# Autodesk Inventor assembly: emsamble caja
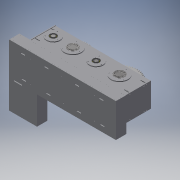
[picture p0: Inventor's stored thumbnail of the model, 180x180]
Saved by Autodesk Inventor 2018 (Build 220112000, 112)
## iProperties
Created: 2017-08-31
Part Number: emsamble caja
Material: Genérico
Document SubType Name: Assembly
Designer: Alumno
Author: Alumno
## Documents named in this file (34)
- C:\Users\isai\Documents\GitHub\caja-reductora-II\emsamble caja.iam
- C:\Users\isai\Documents\GitHub\caja-reductora-II\EJE 2 (30 mm y 15 mm).iam
- C:\Users\isai\Documents\GitHub\caja-reductora-II\TREN 1\Design Accelerator\Engranaje recto12.ipt
- C:\Users\isai\Documents\GitHub\caja-reductora-II\TREN 1\Design Accelerator\Engranaje recto22.ipt
- C:\Users\isai\Documents\GitHub\caja-reductora-II\TREN 2\Design Accelerator\Engranaje recto11.ipt
- C:\Users\isai\Documents\GitHub\caja-reductora-II\TREN 2\Design Accelerator\Engranaje recto21.ipt
- C:\Users\isai\Documents\GitHub\caja-reductora-II\TREN 3\Design Accelerator\Engranaje recto11.ipt
- C:\Users\isai\Documents\GitHub\caja-reductora-II\TREN 3\Design Accelerator\Engranaje recto21.ipt
- C:\Users\isai\Documents\GitHub\caja-reductora-II\EJE 3 (30-45).iam
- C:\Users\isai\Documents\GitHub\caja-reductora-II\EJE 4.iam
- C:\Users\isai\Documents\GitHub\caja-reductora-II\Chaveta- Tren 1.ipt
- C:\Users\isai\Documents\GitHub\caja-reductora-II\Chaveta 25.ipt
- C:\Users\isai\Documents\GitHub\caja-reductora-II\EJE 1.iam
- C:\Users\isai\Documents\GitHub\caja-reductora-II\RODAMIENTO 15 D\6002.iam
- C:\Users\isai\Documents\GitHub\caja-reductora-II\RODAMIENTO 25 D\6005.iam
- C:\Users\isai\Documents\GitHub\caja-reductora-II\ACO.RODA15.ipt
- C:\Users\isai\Documents\GitHub\caja-reductora-II\ACO.RODA25.ipt
- C:\Users\isai\Documents\GitHub\caja-reductora-II\P1.ipt
- C:\Users\isai\Documents\GitHub\caja-reductora-II\P2.ipt
- C:\Users\isai\Documents\GitHub\caja-reductora-II\P3.ipt
- C:\Users\isai\Documents\GitHub\caja-reductora-II\MOTOR DC.ipt
- C:\Users\isai\Documents\Inventor\Content Center Files\R2018\en-US\GB_T 29.1\Bolt GB_T 29.1 M3 x 25.ipt
- C:\Users\isai\Documents\GitHub\caja-reductora-II\SUPORT STEEP.ipt
- C:\Users\isai\Documents\GitHub\caja-reductora-II\SUPORT STEEP 2.ipt
- C:\Users\isai\Documents\Inventor\Content Center Files\R2018\en-US\AS 1112 (2)\AS 1112 - M3  Type 5.ipt
- C:\Users\isai\Documents\Inventor\Content Center Files\R2018\en-US\GB_T 29.1\Bolt GB_T 29.1 M3 x 16.ipt
- C:\Users\isai\Documents\GitHub\caja-reductora-II\PISO.ipt
- C:\Users\isai\Documents\GitHub\caja-reductora-II\FLOOR.ipt
- C:\Users\isai\Documents\GitHub\caja-reductora-II\F1.ipt
- C:\Users\isai\Documents\GitHub\caja-reductora-II\F2.ipt
- C:\Users\isai\Documents\GitHub\caja-reductora-II\F3.ipt
- C:\Users\isai\Documents\GitHub\caja-reductora-II\F4.ipt
- C:\Users\isai\Documents\GitHub\caja-reductora-II\F6.ipt
- C:\Users\isai\Documents\GitHub\caja-reductora-II\F7.ipt
## Components (60 placed, 29 different names)
1. Engranaje recto1:1 — Coincidencia:1, Ángulo:2, Coincidencia:16
2. Engranaje recto2:1 — Coincidencia:5, Coincidencia:6, Ángulo:2, Coincidencia:17
3. Engranaje recto2:2 — Mate:32, Mate:33
4. Engranaje recto1:3 — Mate:27, Mate:30, Mate:40, Mate:51
5. Engranaje recto2:3 — Mate:28, Mate:29
6. EJE 2 (30 mm y 15 mm):3 [sub-assembly] — Coincidencia:2, Coincidencia:3, Coincidencia:4, Coincidencia:5, Ángulo:1, Ángulo:3, Coincidencia:17, Nivelación:1, Mate:31, Mate:34, Mate:36, Mate:41, Mate:44, Mate:56, Mate:59
7. Engranaje recto1:4 — Mate:31, Mate:34, Mate:38, Mate:53
8. EJE 3 (30-45):1 [sub-assembly] — Coincidencia:9, Coincidencia:10, Coincidencia:11, Ángulo:3, Ángulo:4, Nivelación:2, Nivelación:3, Mate:27, Mate:30, Mate:32, Mate:33, Mate:39, Mate:47, Mate:48, Mate:54, Mate:60
9. EJE 4:1 [sub-assembly] — Coincidencia:19, Coincidencia:20, Coincidencia:21, Ángulo:4, Nivelación:3, Mate:28, Mate:29, Mate:42, Mate:43, Mate:49, Mate:55, Mate:57, Mate:61, Mate:64
10. Chaveta- Tren 1:1 — Coincidencia:2, Coincidencia:3, Coincidencia:4, Coincidencia:6
11. Chaveta- Tren 1:2 — Coincidencia:19, Coincidencia:20, Coincidencia:21
12. Chaveta 25:6 — Coincidencia:9, Coincidencia:10, Coincidencia:11
13. EJE 1:1 [sub-assembly] — Coincidencia:1, Ángulo:1, Coincidencia:16, Nivelación:1, Nivelación:2, Mate:35, Mate:45, Mate:46, Mate:50, Mate:52, Mate:58, Mate:63, Mate:89
14. 6002:6 [sub-assembly] — Mate:35, Mate:45, Flush:6
15. 6002:7 [sub-assembly] — Mate:46, Flush:5, Flush:8
16. 6002:8 [sub-assembly] — Mate:36, Mate:38, Flush:9
17. 6002:9 [sub-assembly] — Mate:39, Mate:40, Flush:7
18. 6005:1 [sub-assembly] — Mate:42, Mate:43, Flush:11
19. 6005:2 [sub-assembly] — Mate:47, Mate:48, Flush:4, Flush:5, Flush:12
20. 6005:3 [sub-assembly] — Mate:41, Mate:44, Flush:13
21. 6005:4 [sub-assembly] — Mate:49, Flush:4, Flush:10
22. ACO.RODA15:1 — Mate:50, Flush:6, Mate:62
23. ACO.RODA15:2 — Mate:51, Flush:7
24. ACO.RODA15:3 — Mate:52, Flush:8, Mate:70, Mate:72, Mate:97
25. ACO.RODA15:4 — Mate:53, Flush:9
26. ACO.RODA25:1 — Mate:54, Flush:12
27. ACO.RODA25:2 — Mate:57, Flush:10, Mate:65
28. ACO.RODA25:3 — Mate:56, Flush:13
29. ACO.RODA25:4 — Mate:55, Flush:11
30. P1:1 — Mate:58, Mate:59, Mate:60, Mate:61, Mate:62, Flush:14, Mate:67, Flush:15, Mate:112, Mate:113, Mate:114, Mate:115, Mate:116, Flush:23
31. P2:1 — Mate:63, Mate:64, Mate:65, Mate:66, Mate:71, Mate:73, Mate:74
32. P3:1 — Mate:66, Flush:14, Angle:5
33. P3:2 — Mate:67, Flush:15, Angle:6
34. MOTOR DC:1 — Mate:89, Angle:5, Mate:90, Mate:91
35. Bolt GB/T 29.1 M3x25:2 — Mate:70, Mate:71, Mate:74, Mate:84, Mate:85, Flush:16, Flush:18
36. Bolt GB/T 29.1 M3x25:3 — Mate:72, Mate:73, Mate:75, Mate:86, Flush:17
37. SUPORT STEEP:1 — Mate:75, Mate:84, Mate:88, Mate:99, Mate:100, Mate:101, Mate:102, Mate:104
38. AS 1112 (2) - Metric M3  Type 5:1 — Mate:85, Flush:16, Mate:88
39. AS 1112 (2) - Metric M3  Type 5:2 — Mate:86, Flush:17
40. AS 1112 (2) - Metric M3  Type 5:3 — Mate:98, Flush:19
41. SUPORT STEEP 2:1 — Mate:90, Mate:91, Mate:103, Mate:108, Mate:109, Mate:110, Mate:111
42. Bolt GB/T 29.1 M3x25:4 — Mate:97, Flush:18, Mate:98, Flush:19
43. Bolt GB/T 29.1 M3x25:5 — Mate:99, Mate:101, Mate:107, Flush:22
44. Bolt GB/T 29.1 M3x25:6 — Mate:100, Mate:102, Mate:106, Flush:21
45. Bolt GB/T 29.1 M3x25:7 — Mate:103, Mate:104, Mate:105, Flush:20
46. AS 1112 (2) - Metric M3  Type 5:4 — Mate:105, Flush:20
47. AS 1112 (2) - Metric M3  Type 5:5
48. AS 1112 (2) - Metric M3  Type 5:6 — Mate:106, Flush:21
49. AS 1112 (2) - Metric M3  Type 5:7 — Mate:107, Flush:22
50. Bolt GB/T 29.1 M3x16:1 — Mate:108, Mate:109
51. Bolt GB/T 29.1 M3x16:2 — Mate:110, Mate:111
52. PISO:1 — Mate:112, Mate:113, Mate:114
53. FLOOR:1 — Angle:6, Mate:115, Mate:116, Flush:23, Mate:117, Flush:24, Mate:118, Mate:119, Flush:25, Flush:26, Mate:120, Flush:27, Flush:28, Mate:121, Flush:29, Flush:30, Mate:122, Flush:31, Flush:32, Mate:123, Flush:33, Flush:34
54. F1:1 — Mate:117, Flush:24, Mate:118
55. F2:1 — Mate:119, Flush:25, Flush:26
56. F3:1 — Mate:120, Flush:27, Flush:28
57. F4:1 — Mate:121, Flush:29, Flush:30, Mate:124, Mate:125, Flush:35
58. F6:1 — Mate:122, Flush:31, Flush:32
59. F7:1 — Mate:123, Flush:33, Flush:34
60. FLOOR:2 — Mate:124, Mate:125, Flush:35
## Relationships (137: Mate 96, Flush 35, Angle 6)
- Coincidencia:1 [Mate]: Engranaje recto1:1 ↔ EJE 1:1
- Coincidencia:2 [Mate]: EJE 2 (30 mm y 15 mm):3 ↔ Chaveta- Tren 1:1
- Coincidencia:3 [Mate]: EJE 2 (30 mm y 15 mm):3 ↔ Chaveta- Tren 1:1
- Coincidencia:4 [Mate]: EJE 2 (30 mm y 15 mm):3 ↔ Chaveta- Tren 1:1
- Coincidencia:5 [Mate]: Engranaje recto2:1 ↔ EJE 2 (30 mm y 15 mm):3
- Coincidencia:6 [Mate]: Engranaje recto2:1 ↔ Chaveta- Tren 1:1
- Ángulo:1 [Angle] (0 deg): EJE 2 (30 mm y 15 mm):3 ↔ EJE 1:1
- Ángulo:2 [Angle] (0 deg): Engranaje recto1:1 ↔ Engranaje recto2:1
- Coincidencia:9 [Mate]: EJE 3 (30-45):1 ↔ Chaveta 25:6
- Coincidencia:10 [Mate]: EJE 3 (30-45):1 ↔ Chaveta 25:6
- Coincidencia:11 [Mate]: EJE 3 (30-45):1 ↔ Chaveta 25:6
- Ángulo:3 [Angle] (0 deg): EJE 2 (30 mm y 15 mm):3 ↔ EJE 3 (30-45):1
- Coincidencia:16 [Mate]: Engranaje recto1:1 ↔ EJE 1:1
- Coincidencia:17 [Mate]: Engranaje recto2:1 ↔ EJE 2 (30 mm y 15 mm):3
- Coincidencia:19 [Mate]: EJE 4:1 ↔ Chaveta- Tren 1:2
- Coincidencia:20 [Mate]: EJE 4:1 ↔ Chaveta- Tren 1:2
- Coincidencia:21 [Mate]: EJE 4:1 ↔ Chaveta- Tren 1:2
- Ángulo:4 [Angle] (0 deg): EJE 3 (30-45):1 ↔ EJE 4:1
- Nivelación:1 [Flush]: EJE 2 (30 mm y 15 mm):3 ↔ EJE 1:1
- Nivelación:2 [Flush]: EJE 3 (30-45):1 ↔ EJE 1:1
- Nivelación:3 [Flush]: EJE 3 (30-45):1 ↔ EJE 4:1
- Mate:27: Engranaje recto1:3 ↔ EJE 3 (30-45):1
- Mate:28: Engranaje recto2:3 ↔ EJE 4:1
- Mate:29: Engranaje recto2:3 ↔ EJE 4:1
- Mate:30: Engranaje recto1:3 ↔ EJE 3 (30-45):1
- Mate:31: EJE 2 (30 mm y 15 mm):3 ↔ Engranaje recto1:4
- Mate:32: Engranaje recto2:2 ↔ EJE 3 (30-45):1
- Mate:33: Engranaje recto2:2 ↔ EJE 3 (30-45):1
- Mate:34: EJE 2 (30 mm y 15 mm):3 ↔ Engranaje recto1:4
- Mate:35: EJE 1:1 ↔ 6002:6
- Mate:36: EJE 2 (30 mm y 15 mm):3 ↔ 6002:8
- Mate:38: Engranaje recto1:4 ↔ 6002:8
- Mate:39: EJE 3 (30-45):1 ↔ 6002:9
- Mate:40: Engranaje recto1:3 ↔ 6002:9
- Mate:41: EJE 2 (30 mm y 15 mm):3 ↔ 6005:3
- Mate:42: EJE 4:1 ↔ 6005:1
- Mate:43: EJE 4:1 ↔ 6005:1
- Mate:44: EJE 2 (30 mm y 15 mm):3 ↔ 6005:3
- Mate:45: EJE 1:1 ↔ 6002:6
- Mate:46: EJE 1:1 ↔ 6002:7
- Mate:47: EJE 3 (30-45):1 ↔ 6005:2
- Mate:48: EJE 3 (30-45):1 ↔ 6005:2
- Mate:49: EJE 4:1 ↔ 6005:4
- Flush:4: 6005:2 ↔ 6005:4
- Flush:5: 6002:7 ↔ 6005:2
- Mate:50: EJE 1:1 ↔ ACO.RODA15:1
- Flush:6: 6002:6 ↔ ACO.RODA15:1
- Mate:51: Engranaje recto1:3 ↔ ACO.RODA15:2
- Flush:7: 6002:9 ↔ ACO.RODA15:2
- Mate:52: EJE 1:1 ↔ ACO.RODA15:3
- Flush:8: 6002:7 ↔ ACO.RODA15:3
- Mate:53: Engranaje recto1:4 ↔ ACO.RODA15:4
- Flush:9: 6002:8 ↔ ACO.RODA15:4
- Mate:54: EJE 3 (30-45):1 ↔ ACO.RODA25:1
- Mate:55: EJE 4:1 ↔ ACO.RODA25:4
- Mate:56: EJE 2 (30 mm y 15 mm):3 ↔ ACO.RODA25:3
- Mate:57: EJE 4:1 ↔ ACO.RODA25:2
- Flush:10: 6005:4 ↔ ACO.RODA25:2
- Flush:11: 6005:1 ↔ ACO.RODA25:4
- Flush:12: 6005:2 ↔ ACO.RODA25:1
- Flush:13: 6005:3 ↔ ACO.RODA25:3
- Mate:58: EJE 1:1 ↔ P1:1
- Mate:59: EJE 2 (30 mm y 15 mm):3 ↔ P1:1
- Mate:60: EJE 3 (30-45):1 ↔ P1:1
- Mate:61: EJE 4:1 ↔ P1:1
- Mate:62: ACO.RODA15:1 ↔ P1:1
- Mate:63: EJE 1:1 ↔ P2:1
- Mate:64: EJE 4:1 ↔ P2:1
- Mate:65: ACO.RODA25:2 ↔ P2:1
- Mate:66: P2:1 ↔ P3:1
- Flush:14: P1:1 ↔ P3:1
- Mate:67: P1:1 ↔ P3:2
- Flush:15: P1:1 ↔ P3:2
- Mate:70: ACO.RODA15:3 ↔ Bolt GB/T 29.1 M3x25:2
- Mate:71: P2:1 ↔ Bolt GB/T 29.1 M3x25:2
- Mate:72: ACO.RODA15:3 ↔ Bolt GB/T 29.1 M3x25:3
- Mate:73: P2:1 ↔ Bolt GB/T 29.1 M3x25:3
- Mate:74: P2:1 ↔ Bolt GB/T 29.1 M3x25:2
- Mate:75: Bolt GB/T 29.1 M3x25:3 ↔ SUPORT STEEP:1
- Mate:84: Bolt GB/T 29.1 M3x25:2 ↔ SUPORT STEEP:1
- Mate:85: Bolt GB/T 29.1 M3x25:2 ↔ AS 1112 (2) - Metric M3  Type 5:1
- Flush:16: Bolt GB/T 29.1 M3x25:2 ↔ AS 1112 (2) - Metric M3  Type 5:1
- Mate:86: Bolt GB/T 29.1 M3x25:3 ↔ AS 1112 (2) - Metric M3  Type 5:2
- Flush:17: Bolt GB/T 29.1 M3x25:3 ↔ AS 1112 (2) - Metric M3  Type 5:2
- Mate:88: SUPORT STEEP:1 ↔ AS 1112 (2) - Metric M3  Type 5:1
- Mate:89: EJE 1:1 ↔ MOTOR DC:1
- Angle:5 (0 deg): P3:1 ↔ MOTOR DC:1
- Mate:90: MOTOR DC:1 ↔ SUPORT STEEP 2:1
- Mate:91: MOTOR DC:1 ↔ SUPORT STEEP 2:1
- Mate:97: ACO.RODA15:3 ↔ Bolt GB/T 29.1 M3x25:4
- Flush:18: Bolt GB/T 29.1 M3x25:2 ↔ Bolt GB/T 29.1 M3x25:4
- Mate:98: AS 1112 (2) - Metric M3  Type 5:3 ↔ Bolt GB/T 29.1 M3x25:4
- Flush:19: AS 1112 (2) - Metric M3  Type 5:3 ↔ Bolt GB/T 29.1 M3x25:4
- Mate:99: SUPORT STEEP:1 ↔ Bolt GB/T 29.1 M3x25:5
- Mate:100: SUPORT STEEP:1 ↔ Bolt GB/T 29.1 M3x25:6
- Mate:101: SUPORT STEEP:1 ↔ Bolt GB/T 29.1 M3x25:5
- Mate:102: SUPORT STEEP:1 ↔ Bolt GB/T 29.1 M3x25:6
- Mate:103: SUPORT STEEP 2:1 ↔ Bolt GB/T 29.1 M3x25:7
- Mate:104: SUPORT STEEP:1 ↔ Bolt GB/T 29.1 M3x25:7
- Mate:105: Bolt GB/T 29.1 M3x25:7 ↔ AS 1112 (2) - Metric M3  Type 5:4
- Flush:20: Bolt GB/T 29.1 M3x25:7 ↔ AS 1112 (2) - Metric M3  Type 5:4
- Mate:106: Bolt GB/T 29.1 M3x25:6 ↔ AS 1112 (2) - Metric M3  Type 5:6
- Flush:21: Bolt GB/T 29.1 M3x25:6 ↔ AS 1112 (2) - Metric M3  Type 5:6
- Mate:107: Bolt GB/T 29.1 M3x25:5 ↔ AS 1112 (2) - Metric M3  Type 5:7
- Flush:22: Bolt GB/T 29.1 M3x25:5 ↔ AS 1112 (2) - Metric M3  Type 5:7
- Mate:108: SUPORT STEEP 2:1 ↔ Bolt GB/T 29.1 M3x16:1
- Mate:109: SUPORT STEEP 2:1 ↔ Bolt GB/T 29.1 M3x16:1
- Mate:110: SUPORT STEEP 2:1 ↔ Bolt GB/T 29.1 M3x16:2
- Mate:111: SUPORT STEEP 2:1 ↔ Bolt GB/T 29.1 M3x16:2
- Mate:112: P1:1 ↔ PISO:1
- Mate:113: P1:1 ↔ PISO:1
- Mate:114: P1:1 ↔ PISO:1
- Angle:6 (0 deg): P3:2 ↔ FLOOR:1
- Mate:115: P1:1 ↔ FLOOR:1
- Mate:116: P1:1 ↔ FLOOR:1
- Flush:23: P1:1 ↔ FLOOR:1
- Mate:117: FLOOR:1 ↔ F1:1
- Flush:24: FLOOR:1 ↔ F1:1
- Mate:118: FLOOR:1 ↔ F1:1
- Mate:119: FLOOR:1 ↔ F2:1
- Flush:25: FLOOR:1 ↔ F2:1
- Flush:26: FLOOR:1 ↔ F2:1
- Mate:120: FLOOR:1 ↔ F3:1
- Flush:27: FLOOR:1 ↔ F3:1
- Flush:28: FLOOR:1 ↔ F3:1
- Mate:121: FLOOR:1 ↔ F4:1
- Flush:29: FLOOR:1 ↔ F4:1
- Flush:30: FLOOR:1 ↔ F4:1
- Mate:122: FLOOR:1 ↔ F6:1
- Flush:31: FLOOR:1 ↔ F6:1
- Flush:32: FLOOR:1 ↔ F6:1
- Mate:123: FLOOR:1 ↔ F7:1
- Flush:33: FLOOR:1 ↔ F7:1
- Flush:34: FLOOR:1 ↔ F7:1
- Mate:124: F4:1 ↔ FLOOR:2
- Mate:125: F4:1 ↔ FLOOR:2
- Flush:35: F4:1 ↔ FLOOR:2
